# Autodesk Inventor assembly: bas frame
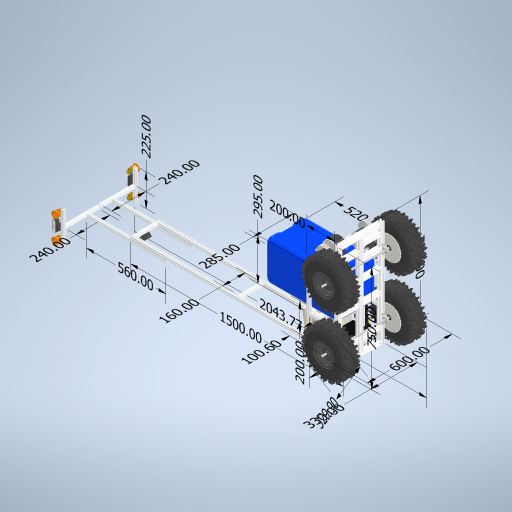
[picture p0: Inventor's stored thumbnail of the model, 512x512]
Saved by Autodesk Inventor 2023 (Build 270158000, 158)
## iProperties
Created: 2023-09-03
Part Number: bas frame
Document SubType Name: Assembly
Designer: sigit
Author: sigit
## Documents named in this file (23)
- D:\Kuliah\SEMESTER 7\Robot Semprot\Design\REVISI2\Assembly\base frame.iam
- D:\Kuliah\SEMESTER 7\Robot Semprot\Design\REVISI2\Part\tslot 3030 750mm.ipt
- D:\Kuliah\SEMESTER 7\Robot Semprot\Design\REVISI2\Part\tslot 3030 270mm.ipt
- D:\Kuliah\SEMESTER 7\Robot Semprot\Design\REVISI2\Part\tslot 3030 690mm.ipt
- D:\Kuliah\SEMESTER 7\Robot Semprot\Design\REVISI2\Part\pillow block 12mm.ipt
- D:\Kuliah\SEMESTER 7\Robot Semprot\Design\REVISI2\Part\poros.ipt
- D:\Kuliah\SEMESTER 7\Robot Semprot\Design\REVISI2\Assembly\roda.iam
- D:\Kuliah\SEMESTER 7\Robot Semprot\Design\REVISI2\Assembly\Motor DC - MY1016Z.iam
- D:\Kuliah\SEMESTER 7\Robot Semprot\Design\REVISI2\Part\tslot 3030 120mm.ipt
- D:\Kuliah\SEMESTER 7\Robot Semprot\Design\REVISI2\Part\sprocket\Roller Chain Sprocket64.ipt
- D:\Kuliah\SEMESTER 7\Robot Semprot\Design\REVISI2\Part\acuan motor.ipt
- D:\Kuliah\SEMESTER 7\Robot Semprot\Design\REVISI2\Part\tslot 2020 200mm.ipt
- D:\Kuliah\SEMESTER 7\Robot Semprot\Design\REVISI2\Part\tslot 2020 295mm.ipt
- D:\Kuliah\SEMESTER 7\Robot Semprot\Design\REVISI2\Part\tslot 2020 280mm.ipt
- D:\Kuliah\SEMESTER 7\Robot Semprot\Design\REVISI2\Assembly\tiangsprayer.iam
- D:\Kuliah\SEMESTER 7\Robot Semprot\Design\2nd ROBOT\Part\2020 219.ipt
- D:\Kuliah\SEMESTER 7\Robot Semprot\Design\REVISI2\Part\pompa\bomba good pump.ipt
- D:\Kuliah\SEMESTER 7\Robot Semprot\Design\2nd ROBOT\Part\jerigenn30L.ipt
- D:\Kuliah\SEMESTER 7\Robot Semprot\Design\2nd ROBOT\Part\Junction Box Assembly.iam
- D:\Kuliah\SEMESTER 7\Robot Semprot\Design\REVISI2\Assembly\nozz.iam
- D:\Kuliah\SEMESTER 7\Robot Semprot\Design\REVISI2\Part\aki\Assembly Inventor\Aki GS GTZ5S.iam
- D:\Kuliah\SEMESTER 7\Robot Semprot\Design\REVISI2\Webcam\Hikvision_DS-U02.iam
- D:\Kuliah\SEMESTER 7\Robot Semprot\Design\REVISI2\Part\holderWebcam.ipt
## Components (62 placed, 22 different names)
1. tslot 3030 750mm:1 — Rotational:1, Rotational:3, Rotational:4, Rotational:11, Rigid:3
2. tslot 3030 750mm:2 — Rotational:2, Rotational:5, Rotational:12, Rotational:13, Rotational:27, Rotational:36
3. tslot 3030 270mm:1 — Rotational:1, Rotational:2
4. tslot 3030 270mm:2 — Rotational:3, Rigid:1, Rotational:30
5. tslot 3030 690mm:1 — Rigid:1, Rotational:37, Rotational:39
6. poros:2 — Rotational:6, Rotational:19, Rotational:21
7. poros:3 — Rotational:7, Rotational:18, Rotational:20
8. tslot 3030 120mm:1 — Rotational:12
9. tslot 3030 120mm:2 — Rotational:11
10. tslot 3030 120mm:4 — Rigid:3, Rotational:24
11. roda:4 [sub-assembly] — Rotational:18
12. roda:5 [sub-assembly] — Rotational:19
13. roda:6 [sub-assembly] — Rotational:21
14. roda:7 [sub-assembly] — Rotational:20
15. Roller Chain Sprocket2:1 — Rotational:22
16. Roller Chain Sprocket2:2 — Rotational:23
17. Motor DC - MY1016Z:1 [sub-assembly] — Rotational:24, Rotational:25
18. Motor DC - MY1016Z:2 [sub-assembly] — Rotational:26
19. acuan motor:1 — Rotational:25, Rotational:26
20. tslot 3030 120mm:7
21. tiangsprayer:1 [sub-assembly] — Rotational:30, Rotational:32, Rigid:4, Rigid:5, Rigid:7, Rigid:8, Rigid:9
22. bomba good pump:1 — Rotational:33
23. bomba good pump:2 — Rotational:35
24. jerigenn30L:1 — Rotational:37
25. Junction Box Assembly:1 [sub-assembly] — Rotational:38
26. Aki GS GTZ5S:1 [sub-assembly] — Rotational:39
27. Hikvision_DS-U02:2 [sub-assembly] — Rigid:7
28. Hikvision_DS-U02:3 [sub-assembly] — Rigid:8
29. holderWebcam:1 — Rigid:9, Rigid:10
30. Hikvision_DS-U02:4 [sub-assembly] — Rigid:10
31. pillow block 12mm:1 — Rotational:4, Rotational:23
32. pillow block 12mm:2 — Rotational:22
33. pillow block 12mm:3 — Rotational:5, Rotational:6
34. pillow block 12mm:4 — Rotational:7
35. tslot 2020 295mm:1 — Rotational:28
36. tslot 2020 295mm:2
37. tslot 2020 280mm:1 — Rotational:29
38. tslot 2020 280mm:2
39. tslot 2020 280mm:3 — Rotational:34
40. tslot 2020 280mm:4
41. nozz:1 [sub-assembly] — Rigid:4
42. nozz:2 [sub-assembly]
43. nozz:3 [sub-assembly]
44. nozz:4 [sub-assembly]
45. nozz:5 [sub-assembly] — Rigid:5
46. nozz:6 [sub-assembly]
47. nozz:7 [sub-assembly]
48. nozz:8 [sub-assembly]
49. tslot 3030 120mm:3 — Rotational:13
50. tslot 3030 120mm:8
51. tslot 2020 200mm:1 — Rotational:27, Rotational:28
52. tslot 2020 200mm:2 — Rotational:29
53. tslot 2020 200mm:3 — Rotational:34
54. tslot 2020 200mm:4
55. 2020 219:1 — Rotational:32, Rotational:33
56. 2020 219:2 — Rotational:35, Rotational:38
57. 2020 219:3
58. 2020 219:4
59. tslot 3030 120mm:9 — Rotational:36
60. tslot 3030 120mm:10
61. tslot 3030 120mm:11
62. tslot 3030 120mm:12
## Component patterns: (2 elements, first: pillow block 12mm:1), (2 elements, first: pillow block 12mm:3), (2 elements), (2 elements), (2 elements, first: tslot 2020 295mm:1), (2 elements, first: tslot 2020 280mm:1), (2 elements), (2 elements, first: tslot 2020 280mm:3), (2 elements), (4 elements, first: nozz:1), (4 elements, first: nozz:5), (2 elements, first: tslot 3030 120mm:3), Component Pattern 3:2 (2 elements), (2 elements, first: tslot 2020 200mm:1), Component Pattern 11:2 (2 elements), (2 elements, first: 2020 219:1), Component Pattern 16:2 (2 elements), (2 elements, first: tslot 3030 120mm:9), Component Pattern 19:2 (2 elements)
## Relationships (39: RevoluteJoint 31, WeldJoint 8)
- Rotational:1 [RevoluteJoint] (-9.486 mm): tslot 3030 750mm:1 ↔ tslot 3030 270mm:1
- Rotational:2 [RevoluteJoint] (9.486 mm): tslot 3030 750mm:2 ↔ tslot 3030 270mm:1
- Rotational:3 [RevoluteJoint] (-9.486 mm): tslot 3030 750mm:1 ↔ tslot 3030 270mm:2
- Rigid:1 [WeldJoint] (-9.486 mm): tslot 3030 270mm:2 ↔ tslot 3030 690mm:1
- Rotational:4 [RevoluteJoint] (9.486 mm): tslot 3030 750mm:1 ↔ pillow block 12mm:1
- Rotational:5 [RevoluteJoint] (9.486 mm): tslot 3030 750mm:2 ↔ pillow block 12mm:3
- Rotational:6 [RevoluteJoint] (460.5 mm): poros:2 ↔ pillow block 12mm:3
- Rotational:7 [RevoluteJoint] (460.5 mm): poros:3 ↔ pillow block 12mm:4
- Rotational:11 [RevoluteJoint] (-9.486 mm): tslot 3030 750mm:1 ↔ tslot 3030 120mm:2
- Rotational:12 [RevoluteJoint] (-9.486 mm): tslot 3030 750mm:2 ↔ tslot 3030 120mm:1
- Rotational:13 [RevoluteJoint] (-9.486 mm): tslot 3030 750mm:2 ↔ tslot 3030 120mm:3
- Rigid:3 [WeldJoint] (9.486 mm): tslot 3030 750mm:1 ↔ tslot 3030 120mm:4
- Rotational:18 [RevoluteJoint] (-123.25 mm): poros:3 ↔ roda:4
- Rotational:19 [RevoluteJoint] (-123.25 mm): poros:2 ↔ roda:5
- Rotational:20 [RevoluteJoint] (-123.25 mm): poros:3 ↔ roda:7
- Rotational:21 [RevoluteJoint] (-123.25 mm): poros:2 ↔ roda:6
- Rotational:22 [RevoluteJoint] (20 mm): Roller Chain Sprocket2:1 ↔ pillow block 12mm:2
- Rotational:23 [RevoluteJoint] (-20 mm): Roller Chain Sprocket2:2 ↔ pillow block 12mm:1
- Rotational:24 [RevoluteJoint] (9.486 mm): tslot 3030 120mm:4 ↔ Motor DC - MY1016Z:1
- Rotational:25 [RevoluteJoint]: Motor DC - MY1016Z:1 ↔ acuan motor:1
- Rotational:26 [RevoluteJoint]: Motor DC - MY1016Z:2 ↔ acuan motor:1
- Rotational:27 [RevoluteJoint] (9.486 mm): tslot 3030 750mm:2 ↔ tslot 2020 200mm:1
- Rotational:28 [RevoluteJoint] (6.1 mm): tslot 2020 295mm:1 ↔ tslot 2020 200mm:1
- Rotational:29 [RevoluteJoint] (6.1 mm): tslot 2020 280mm:1 ↔ tslot 2020 200mm:2
- Rotational:30 [RevoluteJoint] (9.486 mm): tslot 3030 270mm:2 ↔ tiangsprayer:1
- Rotational:32 [RevoluteJoint] (6.1 mm): tiangsprayer:1 ↔ 2020 219:1
- Rotational:33 [RevoluteJoint] (6.1 mm): bomba good pump:1 ↔ 2020 219:1
- Rotational:34 [RevoluteJoint] (6.1 mm): tslot 2020 280mm:3 ↔ tslot 2020 200mm:3
- Rotational:35 [RevoluteJoint] (6.1 mm): bomba good pump:2 ↔ 2020 219:2
- Rotational:36 [RevoluteJoint] (9.486 mm): tslot 3030 750mm:2 ↔ tslot 3030 120mm:9
- Rotational:37 [RevoluteJoint] (4.986 mm): tslot 3030 690mm:1 ↔ jerigenn30L:1
- Rotational:38 [RevoluteJoint] (6.1 mm): Junction Box Assembly:1 ↔ 2020 219:2
- Rigid:4 [WeldJoint]: tiangsprayer:1 ↔ nozz:1
- Rigid:5 [WeldJoint]: tiangsprayer:1 ↔ nozz:5
- Rotational:39 [RevoluteJoint] (9.486 mm): tslot 3030 690mm:1 ↔ Aki GS GTZ5S:1
- Rigid:7 [WeldJoint]: tiangsprayer:1 ↔ Hikvision_DS-U02:2
- Rigid:8 [WeldJoint]: tiangsprayer:1 ↔ Hikvision_DS-U02:3
- Rigid:9 [WeldJoint]: tiangsprayer:1 ↔ holderWebcam:1
- Rigid:10 [WeldJoint]: holderWebcam:1 ↔ Hikvision_DS-U02:4
